# Autodesk Inventor assembly: Full_Design
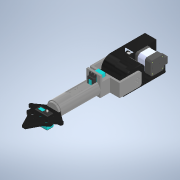
[picture p0: Inventor's stored thumbnail of the model, 180x180]
Saved by Autodesk Inventor 2022 (Build 260153000, 153)
## iProperties
Created: 2022-03-12
Part Number: Full_Design
Document SubType Name: Assembly
Designer: Mlees
Author: Mlees
## Documents named in this file (24)
- C:\Users\Mlees\Desktop\504Engineering\Stepper-Servo_Based_Robotic_Arm\Designs\Version_8\Full_Design.iam
- C:\Users\Mlees\Desktop\504Engineering\Stepper-Servo_Based_Robotic_Arm\Designs\Version_7\Created_Parts\Combined_Gear_Box_Modified_3.ipt
- C:\Users\Mlees\Desktop\504Engineering\Stepper-Servo_Based_Robotic_Arm\Designs\Version_7\Created_Parts\Gear_Cover_modified.ipt
- C:\Users\Mlees\Desktop\504Engineering\Stepper-Servo_Based_Robotic_Arm\Designs\Version_7\Created_Parts\Planet_Carrier_Modifed_with_sun_gear.ipt
- C:\Users\Mlees\Desktop\504Engineering\Stepper-Servo_Based_Robotic_Arm\Designs\Version_7\Created_Parts\Plamet_Carrier.ipt
- C:\Users\Mlees\Desktop\504Engineering\Stepper-Servo_Based_Robotic_Arm\Designs\Version_7\Created_Parts\24_Teeth_Sun_Gear.ipt
- C:\Users\Mlees\Desktop\504Engineering\Stepper-Servo_Based_Robotic_Arm\Designs\Version_7\Created_Parts\36_Teeth_Planet_Gear.ipt
- C:\Users\Mlees\Desktop\504Engineering\Stepper-Servo_Based_Robotic_Arm\Designs\Version_7\Created_Parts\Metal_AttachmentBracket.ipt
- C:\Users\Mlees\Desktop\504Engineering\Stepper-Servo_Based_Robotic_Arm\Designs\Version_7\Created_Parts\Twist_Rod.ipt
- C:\Users\Mlees\Desktop\504Engineering\Stepper-Servo_Based_Robotic_Arm\Designs\Version_8\Downloaded_Parts\9403T15_Tight-Tolerance High-Strength 7075 Aluminum Rod.ipt
- C:\Users\Mlees\Desktop\504Engineering\Stepper-Servo_Based_Robotic_Arm\Designs\Version_8\Downloaded_Parts\GT2 20T Drive Pulley.ipt
- C:\Users\Mlees\Desktop\504Engineering\Stepper-Servo_Based_Robotic_Arm\Designs\Version_8\Downloaded_Parts\GT2 60T Drive Pulley.ipt
- C:\Users\Mlees\Desktop\504Engineering\Stepper-Servo_Based_Robotic_Arm\Designs\Version_8\Downloaded_Parts\124125202-9-stp-mtr-17040w\stp-mtr-17040w.ipt
- C:\Users\Mlees\Desktop\504Engineering\Stepper-Servo_Based_Robotic_Arm\Designs\Version_8\Created_Parts\Combined_Gear_Box_Modified_2.ipt
- C:\Users\Mlees\Desktop\504Engineering\Stepper-Servo_Based_Robotic_Arm\Designs\Version_8\Created_Parts\Tilt_Bracket_Output_2.ipt
- C:\Users\Mlees\Desktop\504Engineering\Stepper-Servo_Based_Robotic_Arm\Designs\Version_8\Created_Parts\Tilt_Bracket_Output_2_Lid.ipt
- C:\Users\Mlees\Desktop\504Engineering\Stepper-Servo_Based_Robotic_Arm\Designs\Version_8\Created_Parts\Twist_Attachment_To_Servo_Horn.ipt
- C:\Users\Mlees\Desktop\504Engineering\Stepper-Servo_Based_Robotic_Arm\Designs\Version_8\Created_Parts\Twist_Servo_Horn.ipt
- C:\Users\Mlees\Desktop\504Engineering\Stepper-Servo_Based_Robotic_Arm\Designs\Version_8\Downloaded_Parts\uploads_files_140274_ServoSW-1211SG.ipt
- C:\Users\Mlees\Desktop\504Engineering\Stepper-Servo_Based_Robotic_Arm\Designs\Version_8\Created_Parts\Claw_Attachment.ipt
- C:\Users\Mlees\Desktop\504Engineering\Stepper-Servo_Based_Robotic_Arm\Designs\Version_8\Created_Parts\Bearing_Side_Tilt.ipt
- C:\Users\Mlees\Desktop\504Engineering\Stepper-Servo_Based_Robotic_Arm\Designs\Version_8\Created_Parts\Tension_Bearings.iam
- C:\Users\Mlees\Desktop\504Engineering\Stepper-Servo_Based_Robotic_Arm\Designs\Version_8\Created_Parts\Claw_Finger.ipt
- C:\Users\Mlees\Desktop\504Engineering\Stepper-Servo_Based_Robotic_Arm\Designs\Version_8\Created_Parts\Claw_Main.ipt
## Components (30 placed, 23 different names)
1. Combined_Gear_Box_Modified_3:1 — Rigid:1, Rigid:4, Rotational:16, Rotational:19, Rotational:20
2. Gear_Cover_modified:1 — Rotational:15
3. Planet_Carrier_Modifed_with_sun_gear:1 — Rotational:4, Rotational:5, Rotational:6, Rotation:2, Rotational:13, Rotational:14
4. Plamet_Carrier:1 — Rotational:7, Rotational:8, Rotational:9, Rotational:14
5. 24_Teeth_Sun_Gear:1 — Rigid:2, Rotation:2, Rotational:13
6. 36_Teeth_Planet_Gear:1 — Rotational:4
7. 36_Teeth_Planet_Gear:2 — Rotational:5
8. 36_Teeth_Planet_Gear:3 — Rotational:6
9. Metal_AttachmentBracket:1 — Rigid:5, Rigid:1
10. 9403T15_Tight-Tolerance High-Strength 7075 Aluminum Rod:1 — Rigid:2, Rigid:3, Rotation:1
11. GT2 20T Drive Pulley:1 — Rotational:2, Rotation:1
12. GT2 60T Drive Pulley:1 — Rigid:3, Rotational:3
13. stp-mtr-17040w:1 — Rigid:5, Rotational:2
14. 36_Teeth_Planet_Gear:4 — Rotational:7
15. 36_Teeth_Planet_Gear:5 — Rotational:8
16. 36_Teeth_Planet_Gear:6 — Rotational:9
17. Combined_Gear_Box_Modified_2:1 — Rigid:4, Rotational:3, Rotational:15
18. Tilt_Bracket_Output_2:1 — Rotational:16, Rigid:9
19. Tilt_Bracket_Output_2_Lid:1 — Rigid:10
20. Twist_Attachment_To_Servo_Horn:1 — Rigid:23, Rotational:21
21. Twist_Rod:1 — Rigid:7, Rigid:23
22. Twist_Servo_Horn:1 — Rotational:18, Rotational:21
23. uploads_files_140274_ServoSW-1211SG:1 — Rigid:9, Rotational:18, Rigid:10
24. Claw_Attachment:1 — Rigid:7, Rigid:11
25. Bearing_Side_Tilt:1 — Rotational:19
26. Tension_Bearings:1 [sub-assembly] — Rotational:20
27. Claw_Finger:1 — Rigid:13
28. Claw_Main:1 — Rigid:11, Rigid:12, Rigid:13, Rigid:14
29. Claw_Finger:2 — Rigid:12
30. uploads_files_140274_ServoSW-1211SG:2 — Rigid:14
## Relationships (31: RevoluteJoint 16, WeldJoint 13, RelateRotation 2)
- Rigid:5 [WeldJoint]: Metal_AttachmentBracket:1 ↔ stp-mtr-17040w:1
- Rigid:1 [WeldJoint]: Combined_Gear_Box_Modified_3:1 ↔ Metal_AttachmentBracket:1
- Rigid:2 [WeldJoint]: 24_Teeth_Sun_Gear:1 ↔ 9403T15_Tight-Tolerance High-Strength 7075 Aluminum Rod:1
- Rigid:3 [WeldJoint]: 9403T15_Tight-Tolerance High-Strength 7075 Aluminum Rod:1 ↔ GT2 60T Drive Pulley:1
- Rigid:4 [WeldJoint]: Combined_Gear_Box_Modified_3:1 ↔ Combined_Gear_Box_Modified_2:1
- Rotational:2 [RevoluteJoint] (5 mm): GT2 20T Drive Pulley:1 ↔ stp-mtr-17040w:1
- Rotational:3 [RevoluteJoint]: GT2 60T Drive Pulley:1 ↔ Combined_Gear_Box_Modified_2:1
- Rotation:1 [RelateRotation] (1 ul): 9403T15_Tight-Tolerance High-Strength 7075 Aluminum Rod:1 ↔ GT2 20T Drive Pulley:1
- Rotational:4 [RevoluteJoint]: Planet_Carrier_Modifed_with_sun_gear:1 ↔ 36_Teeth_Planet_Gear:1
- Rotational:5 [RevoluteJoint]: Planet_Carrier_Modifed_with_sun_gear:1 ↔ 36_Teeth_Planet_Gear:2
- Rotational:6 [RevoluteJoint]: Planet_Carrier_Modifed_with_sun_gear:1 ↔ 36_Teeth_Planet_Gear:3
- Rotational:7 [RevoluteJoint]: Plamet_Carrier:1 ↔ 36_Teeth_Planet_Gear:4
- Rotational:8 [RevoluteJoint]: Plamet_Carrier:1 ↔ 36_Teeth_Planet_Gear:5
- Rotational:9 [RevoluteJoint]: Plamet_Carrier:1 ↔ 36_Teeth_Planet_Gear:6
- Rotation:2 [RelateRotation] (1 ul): Planet_Carrier_Modifed_with_sun_gear:1 ↔ 24_Teeth_Sun_Gear:1
- Rotational:13 [RevoluteJoint]: Planet_Carrier_Modifed_with_sun_gear:1 ↔ 24_Teeth_Sun_Gear:1
- Rotational:14 [RevoluteJoint]: Planet_Carrier_Modifed_with_sun_gear:1 ↔ Plamet_Carrier:1
- Rotational:15 [RevoluteJoint]: Gear_Cover_modified:1 ↔ Combined_Gear_Box_Modified_2:1
- Rotational:16 [RevoluteJoint]: Combined_Gear_Box_Modified_3:1 ↔ Tilt_Bracket_Output_2:1
- Rigid:7 [WeldJoint]: Twist_Rod:1 ↔ Claw_Attachment:1
- Rigid:23 [WeldJoint]: Twist_Attachment_To_Servo_Horn:1 ↔ Twist_Rod:1
- Rigid:9 [WeldJoint]: Tilt_Bracket_Output_2:1 ↔ uploads_files_140274_ServoSW-1211SG:1
- Rotational:18 [RevoluteJoint]: Twist_Servo_Horn:1 ↔ uploads_files_140274_ServoSW-1211SG:1
- Rigid:10 [WeldJoint]: Tilt_Bracket_Output_2_Lid:1 ↔ uploads_files_140274_ServoSW-1211SG:1
- Rotational:19 [RevoluteJoint]: Combined_Gear_Box_Modified_3:1 ↔ Bearing_Side_Tilt:1
- Rotational:20 [RevoluteJoint] (10 mm): Combined_Gear_Box_Modified_3:1 ↔ Tension_Bearings:1
- Rigid:11 [WeldJoint]: Claw_Attachment:1 ↔ Claw_Main:1
- Rigid:12 [WeldJoint]: Claw_Main:1 ↔ Claw_Finger:2
- Rigid:13 [WeldJoint]: Claw_Finger:1 ↔ Claw_Main:1
- Rigid:14 [WeldJoint]: Claw_Main:1 ↔ uploads_files_140274_ServoSW-1211SG:2
- Rotational:21 [RevoluteJoint]: Twist_Attachment_To_Servo_Horn:1 ↔ Twist_Servo_Horn:1
